# Autodesk Inventor assembly: crappy frame that isnt constrained
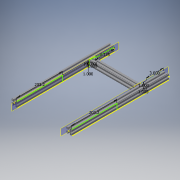
[picture p0: Inventor's stored thumbnail of the model, 180x180]
Saved by Autodesk Inventor 2017 (Build 210142000, 142)
## iProperties
Created: 2017-02-26
Part Number: crappy frame that isnt constrained
Document SubType Name: Assembly
Designer: Jess
Author: Jess
## Documents named in this file (3)
- C:\Users\Jess\Documents\Parts for new robot\crappy frame that isnt constrained.iam
- C:\Users\Jess\Documents\rev extrusion 17 in.ipt
- C:\Users\Jess\Documents\reverend extrusion 9 in.ipt
## Components (3 placed, 2 different names)
1. rev extrusion 17 in:1 — Angle:1, Tangent:1
2. rev extrusion 17 in:2 — Angle:2, Tangent:2
3. reverend extrusion 9 in:1 — Mate:1, Mate:2, Angle:3
## Relationships (8: Angle 3, Mate 3, Tangent 2)
- Angle:1 (0 deg): rev extrusion 17 in:1
- Tangent:1: rev extrusion 17 in:1
- Mate:1: reverend extrusion 9 in:1
- Angle:2 (0 deg): rev extrusion 17 in:2
- Tangent:2: rev extrusion 17 in:2
- Mate:2: reverend extrusion 9 in:1
- Angle:3 (0 deg): reverend extrusion 9 in:1
- Mate:3
